# Autodesk Inventor assembly: centre wing
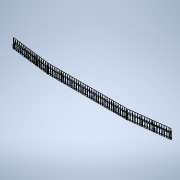
[picture p0: Inventor's stored thumbnail of the model, 180x180]
Saved by Autodesk Inventor 2022 (Build 260153000, 153)
## iProperties
Created: 2021-03-09
Part Number: centre wing
Document SubType Name: Assembly
Designer: Ferdinand Hubbard
Author: Ferdinand Hubbard
## Documents named in this file (4)
- C:\Users\Ferdinand Hubbard\Desktop\solarplane\cad\full wing.iam
- C:\Users\Ferdinand Hubbard\Desktop\solarplane\cad\centre wing section.iam
- C:\Users\Ferdinand Hubbard\Desktop\solarplane\cad\right wing section.iam
- C:\Users\Ferdinand Hubbard\Desktop\solarplane\cad\left wing section.iam
## Components (3 placed, 3 different names)
1. centre wing section:1 [sub-assembly] — Mate:1, Mate:2, Mate:3, Mate:4, Mate:5, Mate:6, Mate:7, Mate:8
2. right wing section:1 [sub-assembly] — Mate:1, Mate:2, Mate:3, Mate:4
3. left wing section:1 [sub-assembly] — Mate:5, Mate:6, Mate:7, Mate:8
## Relationships (8: Mate 8)
- Mate:1: centre wing section:1 ↔ right wing section:1
- Mate:2: centre wing section:1 ↔ right wing section:1
- Mate:3: centre wing section:1 ↔ right wing section:1
- Mate:4: centre wing section:1 ↔ right wing section:1
- Mate:5: centre wing section:1 ↔ left wing section:1
- Mate:6: centre wing section:1 ↔ left wing section:1
- Mate:7: centre wing section:1 ↔ left wing section:1
- Mate:8: centre wing section:1 ↔ left wing section:1
